# Autodesk Inventor assembly: Drilled Wheel
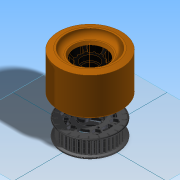
[picture p0: Inventor's stored thumbnail of the model, 180x180]
Saved by Autodesk Inventor 2014 SP2 (Build 180246200, 246)
## iProperties
Created: 2014-05-22
Part Number: Drilled Wheel
Document SubType Name: Assembly
Designer: dliu
Author: dliu
## Documents named in this file (4)
- C:\Users\dliu\Dropbox\dbhome\electric-longboard\dliu\Drilled Wheel tests\Drilled Wheel.iam
- C:\Users\dliu\Dropbox\dbhome\electric-longboard\dliu\Pulleys\217-3199-STEP.iam
- C:\Users\dliu\Dropbox\dbhome\electric-longboard\dliu\Wheel Blank Pro 83mm.ipt
- C:\Users\dliu\Dropbox\dbhome\electric-longboard\dliu\drill sketch.ipt
## Components (3 placed, 3 different names)
1. 217-3199-STEP:1 [sub-assembly] — Mate:2, Mate:5, Mate:6
2. Wheel Blank Pro 83mm:1 — Mate:1, Mate:3, Mate:4, Mate:6
3. drill sketch:1 — Flush:1
## Relationships (7: Mate 6, Flush 1)
- Mate:1: Wheel Blank Pro 83mm:1
- Mate:2: 217-3199-STEP:1
- Mate:3: Wheel Blank Pro 83mm:1
- Mate:4: Wheel Blank Pro 83mm:1
- Flush:1: drill sketch:1
- Mate:5: 217-3199-STEP:1
- Mate:6 (101.6 mm): 217-3199-STEP:1 ↔ Wheel Blank Pro 83mm:1
